# Autodesk Inventor assembly: robot3
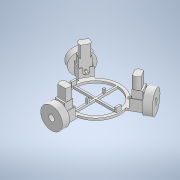
[picture p0: Inventor's stored thumbnail of the model, 180x180]
Saved by Autodesk Inventor 2020 (Build 240168000, 168)
## iProperties
Created: 2020-03-23
Part Number: robot3
Document SubType Name: Assembly
Designer: Tarsoly
Author: Tarsoly
## Documents named in this file (4)
- D:\Users\Tarsoly\Dokumentumok\BME\8. Félév\Önlab\3d\robot3.iam
- D:\Users\Tarsoly\Dokumentumok\BME\8. Félév\Önlab\3d\bottom3.ipt
- D:\Users\Tarsoly\Dokumentumok\BME\8. Félév\Önlab\3d\motor3.ipt
- D:\Users\Tarsoly\Dokumentumok\BME\8. Félév\Önlab\3d\omniwheel.ipt
## Components (7 placed, 3 different names)
1. bottom3:1 — Mate:1, Flush:1, Flush:2, Mate:2, Mate:3, Mate:4, Mate:5, Mate:6, Mate:7, Mate:8, Mate:9, Mate:10, Mate:14, Mate:15, Mate:16
2. motor3:1 — Mate:2, Mate:3, Mate:4, Mate:11
3. omniwheel:1 — Mate:11, Mate:14
4. motor3:2 — Mate:5, Mate:6, Mate:7, Mate:12
5. omniwheel:2 — Mate:12, Mate:16
6. motor3:3 — Mate:8, Mate:9, Mate:10, Mate:13
7. omniwheel:3 — Mate:13, Mate:15
## Relationships (18: Mate 16, Flush 2)
- Mate:1: bottom3:1
- Flush:1 (-2 mm): bottom3:1
- Flush:2 (-2 mm): bottom3:1
- Mate:2: bottom3:1 ↔ motor3:1
- Mate:3: bottom3:1 ↔ motor3:1
- Mate:4 (1 mm): bottom3:1 ↔ motor3:1
- Mate:5 (1 mm): bottom3:1 ↔ motor3:2
- Mate:6: bottom3:1 ↔ motor3:2
- Mate:7: bottom3:1 ↔ motor3:2
- Mate:8: bottom3:1 ↔ motor3:3
- Mate:9 (1 mm): bottom3:1 ↔ motor3:3
- Mate:10: bottom3:1 ↔ motor3:3
- Mate:11: motor3:1 ↔ omniwheel:1
- Mate:12: motor3:2 ↔ omniwheel:2
- Mate:13: motor3:3 ↔ omniwheel:3
- Mate:14 (1 mm): bottom3:1 ↔ omniwheel:1
- Mate:15 (1 mm): bottom3:1 ↔ omniwheel:3
- Mate:16 (1 mm): bottom3:1 ↔ omniwheel:2
